# Autodesk Inventor assembly: Claw_Assembly
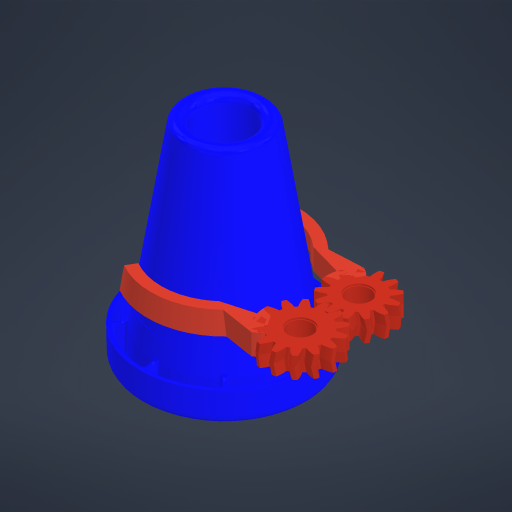
[picture p0: Inventor's stored thumbnail of the model, 512x512]
Saved by Autodesk Inventor 2024.2 (Build 282272000, 272)
## iProperties
Created: 2024-06-17
Part Number: Claw_Assembly
Document SubType Name: Assembly
Designer: warm
Author: warm
## Documents named in this file (4)
- C:\Users\warm\Desktop\Robotics\Cad\Powerplay_Fun\Parts\Claw_Assembly.iam
- C:\Users\warm\Desktop\Robotics\Cad\Powerplay_Fun\Parts\Intake_Claw.ipt
- C:\Users\warm\Desktop\Robotics\Cad\Powerplay_Fun\Parts\Claw_Assembly\Design Accelerator\Spur Gears2.iam
- C:\Users\warm\Desktop\Robotics\Cad\Powerplay_Fun\Parts\Claw_Assembly\Design Accelerator\Spur Gears2_MIR.iam
## Components (3 placed, 3 different names)
1. Intake_Claw:1 — Angle:1, Flush:1, Flush:2, Flush:3
2. Spur Gears:1 [sub-assembly] — Mate:1, Mate:2, Mate:3, Angle:1, Flush:2, Flush:3
3. Spur Gears2_MIR:1 [sub-assembly] — Mate:1, Mate:2, Mate:3, Flush:1
## Relationships (7: Mate 3, Flush 3, Angle 1)
- Mate:1: Spur Gears:1 ↔ Spur Gears2_MIR:1
- Mate:2: Spur Gears:1 ↔ Spur Gears2_MIR:1
- Mate:3: Spur Gears:1 ↔ Spur Gears2_MIR:1
- Angle:1 (0 deg): Intake_Claw:1 ↔ Spur Gears:1
- Flush:1: Intake_Claw:1 ↔ Spur Gears2_MIR:1
- Flush:2: Intake_Claw:1 ↔ Spur Gears:1
- Flush:3: Intake_Claw:1 ↔ Spur Gears:1
